# Autodesk Inventor assembly: case_assembly
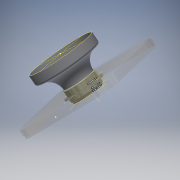
[picture p0: Inventor's stored thumbnail of the model, 180x180]
Saved by Autodesk Inventor 2019 (Build 230136000, 136)
## iProperties
Created: 2019-01-02
Part Number: case_assembly
Document SubType Name: Assembly
Designer: jmc
Author: jmc
## Documents named in this file (17)
- D:\Inventor\Projects\CatFeeder\version2 (fixed enclosure)\version2_newcone.iam
- D:\Inventor\Projects\CatFeeder\Case\version2\case.ipt
- D:\Inventor\Projects\3party\Boards\ArduinoNano\arduino nano.iam
- D:\Inventor\Projects\3party\Boards\Raspberry Pi 3\Raspberry Pi 3.ipt
- D:\Inventor\Projects\3party\Trasformer\Transformer.ipt
- D:\Inventor\Projects\CatFeeder\Case\version2\case_top.ipt
- D:\Inventor\Projects\CatFeeder\Case\version2\case_bottom.ipt
- D:\Inventor\Projects\CatFeeder\Case\version2\Pata.ipt
- D:\Inventor\Projects\CatFeeder\Case\version2\pata_macho.ipt
- D:\Inventor\Projects\CatFeeder\JarCone\version2\cono_nuevo.ipt
- D:\Inventor\Projects\CatFeeder\JarCone\version2\adaptador_cono.ipt
- D:\Inventor\Projects\CatFeeder\Jar\Jar.ipt
- D:\Inventor\Projects\3party\Servos\MG995.ipt
- D:\Inventor\Projects\CatFeeder\Trap\version2\trapdoor_servo.ipt
- D:\Inventor\Projects\CatFeeder\Ramp\version2\ramp.ipt
- D:\Inventor\Projects\CatFeeder\Ramp\version2\ramp_adapter.ipt
- D:\Inventor\Projects\CatFeeder\ServoHolder\servoholder.ipt
## Components (22 placed, 16 different names)
1. case:1
2. case_top:1 — Rigid:16
3. cono_nuevo:1 — Rigid:12, Rigid:13
4. adaptador_cono:1 — Rigid:13, Rotational:6, Rigid:16
5. Jar:1 — Rigid:12
6. case_bottom:1 — Rigid:1, Rigid:3, Rigid:4, Flush:1, Rotational:1, Rigid:6, Rigid:7, Rigid:8, Flush:12, Flush:17, Flush:19
7. trapdoor_servo:1 — Rotational:6, Rotational:7
8. MG995:1 — Rotational:7, Flush:16, Flush:18
9. ramp:1 — Flush:12, Flush:16, Flush:19
10. servoholder:1 — Flush:18
11. ramp_adapter:1 — Flush:17
12. arduino nano:1 [sub-assembly] — Rigid:4
13. Raspberry Pi 3:1 — Rigid:1
14. Transformer:1 — Rigid:3
15. pata_macho:4 — Rotational:5
16. pata_macho:3 — Rotational:3
17. pata_macho:2 — Rotational:4
18. pata_macho:1 — Rotational:2
19. Pata:1 — Flush:1, Rotational:1, Rotational:2
20. Pata:2 — Rigid:8, Rotational:5
21. Pata:3 — Rigid:7, Rotational:3
22. Pata:4 — Rigid:6, Rotational:4
## Relationships (22: WeldJoint 9, RevoluteJoint 7, Flush 6)
- Rigid:1 [WeldJoint]: case_bottom:1 ↔ Raspberry Pi 3:1
- Rigid:3 [WeldJoint]: case_bottom:1 ↔ Transformer:1
- Rigid:4 [WeldJoint]: case_bottom:1 ↔ arduino nano:1
- Flush:1: case_bottom:1 ↔ Pata:1
- Rotational:1 [RevoluteJoint]: case_bottom:1 ↔ Pata:1
- Rigid:6 [WeldJoint]: case_bottom:1 ↔ Pata:4
- Rigid:7 [WeldJoint]: case_bottom:1 ↔ Pata:3
- Rigid:8 [WeldJoint]: case_bottom:1 ↔ Pata:2
- Rotational:2 [RevoluteJoint]: pata_macho:1 ↔ Pata:1
- Rotational:3 [RevoluteJoint]: pata_macho:3 ↔ Pata:3
- Rotational:4 [RevoluteJoint]: pata_macho:2 ↔ Pata:4
- Rotational:5 [RevoluteJoint]: pata_macho:4 ↔ Pata:2
- Rigid:12 [WeldJoint]: cono_nuevo:1 ↔ Jar:1
- Rigid:13 [WeldJoint]: cono_nuevo:1 ↔ adaptador_cono:1
- Rotational:6 [RevoluteJoint] (0.4 mm): adaptador_cono:1 ↔ trapdoor_servo:1
- Rotational:7 [RevoluteJoint]: trapdoor_servo:1 ↔ MG995:1
- Flush:12: case_bottom:1 ↔ ramp:1
- Flush:16: MG995:1 ↔ ramp:1
- Flush:17: case_bottom:1 ↔ ramp_adapter:1
- Flush:18: MG995:1 ↔ servoholder:1
- Flush:19: case_bottom:1 ↔ ramp:1
- Rigid:16 [WeldJoint]: case_top:1 ↔ adaptador_cono:1
## Named parameters: HOLE_TOLERANCE = 0.15 mm, CASE_TOLERANCE = 0.08 mm
